# Autodesk Inventor assembly: Assembly1
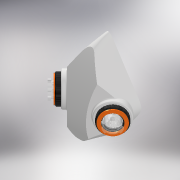
[picture p0: Inventor's stored thumbnail of the model, 180x180]
Saved by Autodesk Inventor 2021 (Build 250183000, 183)
## iProperties
Created: 2020-06-11
Part Number: Assembly1
Document SubType Name: Assembly
Designer: Derm
Author: Derm
## Documents named in this file (5)
- C:\Users\Derm\n95\v7\Assembly1.iam
- C:\Users\Derm\n95\v7\maskBody.ipt
- C:\Users\Derm\n95\v7\3dpBayonetteMountV2.ipt
- C:\Users\Derm\n95\v7\3dpBayonetteMountV1Fastener.ipt
- C:\Users\Derm\n95\v7\outerMountGasket.ipt
## Components (7 placed, 4 different names)
1. maskBody:1 — Mate:1, Mate:2, Mate:3, Mate:5, Mate:6, Mate:7
2. 3dpBayonetteMountV2:1 — Mate:5, Mate:6, Mate:8, Mate:9
3. 3dpBayonetteMountV1Fastener:1 — Mate:3, Mate:4, Mate:12
4. outerMountGasket:1 — Mate:9, Mate:11
5. outerMountGasket:2 — Mate:10, Mate:12
6. 3dpBayonetteMountV2:2 — Mate:1, Mate:2, Mate:4, Mate:10
7. 3dpBayonetteMountV1Fastener:2 — Mate:7, Mate:8, Mate:11
## Relationships (12: Mate 12)
- Mate:1: maskBody:1 ↔ 3dpBayonetteMountV2:2
- Mate:2: maskBody:1 ↔ 3dpBayonetteMountV2:2
- Mate:3: maskBody:1 ↔ 3dpBayonetteMountV1Fastener:1
- Mate:4: 3dpBayonetteMountV1Fastener:1 ↔ 3dpBayonetteMountV2:2
- Mate:5: maskBody:1 ↔ 3dpBayonetteMountV2:1
- Mate:6: maskBody:1 ↔ 3dpBayonetteMountV2:1
- Mate:7: maskBody:1 ↔ 3dpBayonetteMountV1Fastener:2
- Mate:8: 3dpBayonetteMountV2:1 ↔ 3dpBayonetteMountV1Fastener:2
- Mate:9: 3dpBayonetteMountV2:1 ↔ outerMountGasket:1
- Mate:10: outerMountGasket:2 ↔ 3dpBayonetteMountV2:2
- Mate:11: outerMountGasket:1 ↔ 3dpBayonetteMountV1Fastener:2
- Mate:12: 3dpBayonetteMountV1Fastener:1 ↔ outerMountGasket:2
